# Autodesk Inventor assembly: Mark2
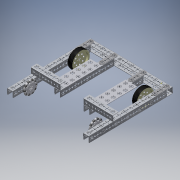
[picture p0: Inventor's stored thumbnail of the model, 180x180]
Saved by Autodesk Inventor 2017 (Build 210142000, 142)
## iProperties
Created: 2016-09-25
Part Number: Mark2
Document SubType Name: Assembly
Designer: Spartacles
Author: Spartacles
## Documents named in this file (11)
- C:\Users\Spartacles\Desktop\FTC Parts\2016launcher\Mark2.iam
- C:\Users\Spartacles\Desktop\FTC Parts\2016launcher\UTubes\Star3Tube.ipt
- C:\Users\Spartacles\Desktop\FTC Parts\2016launcher\UTubes\Star5Tube.ipt
- C:\Users\Spartacles\Desktop\FTC Parts\2016launcher\UTubes\Star7Tube.ipt
- C:\Users\Spartacles\Desktop\FTC Parts\Axle Hub\Axle hub.ipt
- C:\Users\Spartacles\Desktop\FTC Parts\Axel\Axel.ipt
- C:\Users\Spartacles\Desktop\FTC Parts\BlackWheels\4 Inch Wheel.ipt
- C:\Users\Spartacles\Desktop\FTC Parts\omni\3inch OmniWheel.iam
- C:\Users\Spartacles\Documents\Pitsco Education-739273\Pitsco Education-739273.ipt
- C:\Users\Spartacles\Documents\Pitsco Education-739272 (1)\Pitsco Education-739272.ipt
- C:\Users\Spartacles\Documents\Pitsco Education-739073\Pitsco Education-739073.ipt
## Components (32 placed, 10 different names)
1. Star5Tube:1 — Mate:6, Flush:12, Flush:13, Mate:74, Mate:75, Mate:76, Mate:105, Mate:106, Mate:107
2. Star5Tube:2 — Flush:7, Flush:8, Mate:61, Mate:79, Mate:81, Mate:94, Mate:108, Mate:109, Mate:110
3. Star7Tube:1 — Mate:4, Flush:6, Flush:9, Mate:17, Mate:18, Mate:20, Mate:24, Mate:25, Mate:32, Mate:44, Flush:26, Mate:64, Mate:65, Mate:66
4. Star7Tube:2 — Flush:11, Flush:14, Mate:8, Mate:9, Mate:13, Mate:30, Mate:31, Mate:33, Mate:36, Mate:45, Mate:67, Mate:70, Mate:71
5. Star3Tube:1 — Mate:4, Flush:6, Flush:7, Flush:8, Flush:9, Mate:44, Flush:26, Mate:61
6. Star3Tube:2 — Mate:6, Flush:11, Flush:12, Flush:13, Flush:14, Mate:36, Mate:45
7. Axle hub:1 — Mate:19, Mate:20
8. Axle hub:2 — Mate:14, Mate:15, Mate:16, Mate:18
9. Axle hub:3 — Mate:12, Mate:13
10. Axle hub:4 — Mate:7, Mate:8, Mate:9, Mate:10, Mate:11
11. Axel:1 — Mate:16, Flush:16, Mate:17, Mate:19
12. Axel:2 — Mate:27, Flush:18, Mate:30, Mate:34
13. Axel:3 — Mate:23, Flush:17, Mate:26
14. Axel:4 — Mate:7, Flush:15, Mate:12
15. 4 Inch Wheel:1 — Mate:21, Mate:22, Flush:17
16. 4 Inch Wheel:2 — Mate:28, Mate:29, Flush:18
17. 3inch OmniWheel:1 [sub-assembly] — Mate:10, Mate:11, Flush:15
18. 3inch OmniWheel:2 [sub-assembly] — Mate:14, Mate:15, Flush:16
19. Axle hub:5 — Mate:21, Mate:22, Mate:23, Mate:24, Mate:32
20. Axle hub:6 — Mate:25, Mate:26
21. Axle hub:7 — Mate:27, Mate:28, Mate:29, Mate:31
22. Axle hub:8 — Mate:33, Mate:34
23. Star3Tube:3 — Mate:88, Mate:89, Mate:90, Mate:98, Mate:99, Mate:100, Mate:101, Mate:102, Mate:103
24. Star5Tube:3 — Mate:91, Mate:92, Mate:93, Mate:95, Mate:96, Mate:97, Mate:104
25. Pitsco Education-739273:1 — Mate:67, Mate:70, Mate:71, Mate:95, Mate:96
26. Pitsco Education-739273:2 — Mate:79, Mate:81, Mate:94, Mate:98, Mate:100
27. Pitsco Education-739273:3 — Mate:74, Mate:75, Mate:76, Mate:97
28. Pitsco Education-739273:4 — Mate:64, Mate:65, Mate:66, Mate:99
29. Pitsco Education-739272:1 — Mate:88, Mate:89, Mate:90, Mate:91, Mate:92, Mate:93
30. Pitsco Education-739272:2 — Mate:101, Mate:102, Mate:103, Mate:104
31. Pitsco Education-739073:1 — Mate:108, Mate:109, Mate:110
32. Pitsco Education-739073:3 — Mate:105, Mate:106, Mate:107
## Relationships (82: Mate 69, Flush 13)
- Mate:4: Star7Tube:1 ↔ Star3Tube:1
- Flush:6: Star7Tube:1 ↔ Star3Tube:1
- Flush:7: Star5Tube:2 ↔ Star3Tube:1
- Flush:8: Star5Tube:2 ↔ Star3Tube:1
- Flush:9: Star7Tube:1 ↔ Star3Tube:1
- Mate:6: Star5Tube:1 ↔ Star3Tube:2
- Flush:11: Star7Tube:2 ↔ Star3Tube:2
- Flush:12: Star5Tube:1 ↔ Star3Tube:2
- Flush:13: Star5Tube:1 ↔ Star3Tube:2
- Flush:14: Star7Tube:2 ↔ Star3Tube:2
- Mate:7: Axle hub:4 ↔ Axel:4
- Mate:8: Star7Tube:2 ↔ Axle hub:4
- Mate:9: Star7Tube:2 ↔ Axle hub:4
- Mate:10: Axle hub:4 ↔ 3inch OmniWheel:1
- Mate:11: Axle hub:4 ↔ 3inch OmniWheel:1
- Flush:15: Axel:4 ↔ 3inch OmniWheel:1
- Mate:12: Axle hub:3 ↔ Axel:4
- Mate:13: Star7Tube:2 ↔ Axle hub:3
- Mate:14: Axle hub:2 ↔ 3inch OmniWheel:2
- Mate:15: Axle hub:2 ↔ 3inch OmniWheel:2
- Mate:16: Axle hub:2 ↔ Axel:1
- Flush:16: Axel:1 ↔ 3inch OmniWheel:2
- Mate:17: Star7Tube:1 ↔ Axel:1
- Mate:18: Star7Tube:1 ↔ Axle hub:2
- Mate:19: Axle hub:1 ↔ Axel:1
- Mate:20: Star7Tube:1 ↔ Axle hub:1
- Mate:21: 4 Inch Wheel:1 ↔ Axle hub:5
- Mate:22: 4 Inch Wheel:1 ↔ Axle hub:5
- Mate:23: Axel:3 ↔ Axle hub:5
- Flush:17: Axel:3 ↔ 4 Inch Wheel:1
- Mate:24: Star7Tube:1 ↔ Axle hub:5
- Mate:25: Star7Tube:1 ↔ Axle hub:6
- Mate:26: Axel:3 ↔ Axle hub:6
- Mate:27: Axel:2 ↔ Axle hub:7
- Mate:28: 4 Inch Wheel:2 ↔ Axle hub:7
- Mate:29: 4 Inch Wheel:2 ↔ Axle hub:7
- Flush:18: Axel:2 ↔ 4 Inch Wheel:2
- Mate:30: Star7Tube:2 ↔ Axel:2
- Mate:31 (6.35 mm): Star7Tube:2 ↔ Axle hub:7
- Mate:32 (6.35 mm): Star7Tube:1 ↔ Axle hub:5
- Mate:33: Star7Tube:2 ↔ Axle hub:8
- Mate:34: Axel:2 ↔ Axle hub:8
- Mate:36: Star7Tube:2 ↔ Star3Tube:2
- Mate:44: Star7Tube:1 ↔ Star3Tube:1
- Flush:26: Star7Tube:1 ↔ Star3Tube:1
- Mate:45: Star7Tube:2 ↔ Star3Tube:2
- Mate:52 (0.2794 mm)
- Mate:61: Star5Tube:2 ↔ Star3Tube:1
- Mate:64: Star7Tube:1 ↔ Pitsco Education-739273:4
- Mate:65: Star7Tube:1 ↔ Pitsco Education-739273:4
- Mate:66: Star7Tube:1 ↔ Pitsco Education-739273:4
- Mate:67: Star7Tube:2 ↔ Pitsco Education-739273:1
- Mate:70: Star7Tube:2 ↔ Pitsco Education-739273:1
- Mate:71: Star7Tube:2 ↔ Pitsco Education-739273:1
- Mate:74: Star5Tube:1 ↔ Pitsco Education-739273:3
- Mate:75: Star5Tube:1 ↔ Pitsco Education-739273:3
- Mate:76: Star5Tube:1 ↔ Pitsco Education-739273:3
- Mate:79: Star5Tube:2 ↔ Pitsco Education-739273:2
- Mate:81: Star5Tube:2 ↔ Pitsco Education-739273:2
- Mate:88: Star3Tube:3 ↔ Pitsco Education-739272:1
- Mate:89: Star3Tube:3 ↔ Pitsco Education-739272:1
- Mate:90: Star3Tube:3 ↔ Pitsco Education-739272:1
- Mate:91: Star5Tube:3 ↔ Pitsco Education-739272:1
- Mate:92: Star5Tube:3 ↔ Pitsco Education-739272:1
- Mate:93: Star5Tube:3 ↔ Pitsco Education-739272:1
- Mate:94: Star5Tube:2 ↔ Pitsco Education-739273:2
- Mate:95: Star5Tube:3 ↔ Pitsco Education-739273:1
- Mate:96: Star5Tube:3 ↔ Pitsco Education-739273:1
- Mate:97: Star5Tube:3 ↔ Pitsco Education-739273:3
- Mate:98: Star3Tube:3 ↔ Pitsco Education-739273:2
- Mate:99: Star3Tube:3 ↔ Pitsco Education-739273:4
- Mate:100: Star3Tube:3 ↔ Pitsco Education-739273:2
- Mate:101: Star3Tube:3 ↔ Pitsco Education-739272:2
- Mate:102: Star3Tube:3 ↔ Pitsco Education-739272:2
- Mate:103: Star3Tube:3 ↔ Pitsco Education-739272:2
- Mate:104: Star5Tube:3 ↔ Pitsco Education-739272:2
- Mate:105: Star5Tube:1 ↔ Pitsco Education-739073:3
- Mate:106: Star5Tube:1 ↔ Pitsco Education-739073:3
- Mate:107: Star5Tube:1 ↔ Pitsco Education-739073:3
- Mate:108: Star5Tube:2 ↔ Pitsco Education-739073:1
- Mate:109: Star5Tube:2 ↔ Pitsco Education-739073:1
- Mate:110: Star5Tube:2 ↔ Pitsco Education-739073:1
